# Autodesk Inventor assembly: Assieme_Disco
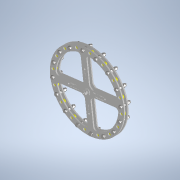
[picture p0: Inventor's stored thumbnail of the model, 180x180]
Saved by Autodesk Inventor 2020.2 (Build 242310000, 310)
## iProperties
Created: 2019-12-29
Part Number: Assieme_Disco
Document SubType Name: Assembly
Designer: socci
Mass: 580.168 g
Surface Area: 1810.87 cm^2
Volume: 239.955 cm^3
Density: 2.41782 g/cm^3
Author: socci
## Documents named in this file (8)
- C:\Users\socci\Desktop\mv-Project\04_PartDraw\Assieme_Disco.iam
- C:\Users\socci\Desktop\04_PartDraw\Componenti\24_Disco.ipt
- C:\Users\socci\Desktop\mv-Project\04_PartDraw\Componenti\26_Collana_di_Sfere.ipt
- C:\Users\socci\Documents\Inventor\Content Center Files\R2020\it-IT\DIN 1587\DIN 1587 - M6 x 1.ipt
- C:\Users\socci\Documents\Inventor\Content Center Files\R2020\it-IT\DIN 934\DIN 934 - M6 x 1.ipt
- C:\Users\socci\Desktop\mv-Project\04_PartDraw\Componenti\28_Rondella_M6.ipt
- C:\Users\socci\Documents\Inventor\Content Center Files\R2020\it-IT\DIN 933\DIN 933 - M6  x 30.ipt
- C:\Users\socci\Desktop\mv-Project\04_PartDraw\Componenti\9_Flangia.ipt
## Components (148 placed, 7 different names)
1. 24_Disco:1 — Inserimento:1, Inserimento:2, Inserimento:3, Inserimento:4
2. 24_Disco:2 — Inserimento:1, Inserimento:2, Inserimento:3, Inserimento:4, Coincidente:1, Coincidente:2, Inserimento:21, Inserimento:134, Inserimento:135, Coincidente:3, Inserimento:136, Inserimento:137, Inserimento:138, Inserimento:139, Inserimento:140, Inserimento:141, Inserimento:142, Inserimento:143, Inserimento:144, Inserimento:145, Inserimento:146, Inserimento:147, Inserimento:148, Coincidente:4, Inserimento:149, Inserimento:150
3. 26_Collana_di_Sfere:1 — Coincidente:1, Coincidente:2
4. DIN 933 - sostituito da DIN EN 24017 M6  x 30:1 — Inserimento:5
5. DIN 934 - sostituito da DIN EN 24032/28673/28674 M6:1 — Inserimento:7, Inserimento:8
6. 28_Rondella_M6:1 — Inserimento:5, Inserimento:6, Inserimento:134
7. 28_Rondella_M6:2 — Inserimento:6, Inserimento:7
8. 28_Rondella_M6:3 — Inserimento:8, Inserimento:9
9. 28_Rondella_M6:4 — Inserimento:11, Inserimento:12
10. 28_Rondella_M6:5 — Inserimento:9, Inserimento:10
11. 28_Rondella_M6:6 — Inserimento:10, Inserimento:11
12. DIN 1587 M6:1 — Inserimento:12
13. DIN 1587 M6:2
14. DIN 934 - sostituito da DIN EN 24032/28673/28674 M6:2
15. 28_Rondella_M6:7 — Inserimento:21
16. DIN 933 - sostituito da DIN EN 24017 M6  x 30:2
17. 28_Rondella_M6:8
18. 28_Rondella_M6:9
19. 28_Rondella_M6:10
20. 28_Rondella_M6:11
21. 28_Rondella_M6:12
22. DIN 1587 M6:3
23. DIN 934 - sostituito da DIN EN 24032/28673/28674 M6:3
24. 28_Rondella_M6:13 — Inserimento:147
25. DIN 933 - sostituito da DIN EN 24017 M6  x 30:3
26. 28_Rondella_M6:14
27. 28_Rondella_M6:15
28. 28_Rondella_M6:16
29. 28_Rondella_M6:17
30. 28_Rondella_M6:18
31. DIN 1587 M6:4
32. DIN 934 - sostituito da DIN EN 24032/28673/28674 M6:4
33. 28_Rondella_M6:19 — Inserimento:136
34. DIN 933 - sostituito da DIN EN 24017 M6  x 30:4
35. 28_Rondella_M6:20
36. 28_Rondella_M6:21
37. 28_Rondella_M6:22
38. 28_Rondella_M6:23
39. 28_Rondella_M6:24
40. DIN 1587 M6:5
41. DIN 934 - sostituito da DIN EN 24032/28673/28674 M6:5
42. 28_Rondella_M6:25 — Inserimento:146
43. DIN 933 - sostituito da DIN EN 24017 M6  x 30:5
44. 28_Rondella_M6:26
45. 28_Rondella_M6:27
46. 28_Rondella_M6:28
47. 28_Rondella_M6:29
48. 28_Rondella_M6:30
49. DIN 1587 M6:6
50. DIN 934 - sostituito da DIN EN 24032/28673/28674 M6:6
51. 28_Rondella_M6:31 — Inserimento:148
52. DIN 933 - sostituito da DIN EN 24017 M6  x 30:6
53. 28_Rondella_M6:32
54. 28_Rondella_M6:33
55. 28_Rondella_M6:34
56. 28_Rondella_M6:35
57. 28_Rondella_M6:36
58. DIN 1587 M6:7
59. DIN 934 - sostituito da DIN EN 24032/28673/28674 M6:7
60. 28_Rondella_M6:37 — Inserimento:144
61. DIN 933 - sostituito da DIN EN 24017 M6  x 30:7
62. 28_Rondella_M6:38
63. 28_Rondella_M6:39
64. 28_Rondella_M6:40
65. 28_Rondella_M6:41
66. 28_Rondella_M6:42
67. DIN 1587 M6:8
68. DIN 934 - sostituito da DIN EN 24032/28673/28674 M6:8
69. 28_Rondella_M6:43 — Inserimento:137
70. DIN 933 - sostituito da DIN EN 24017 M6  x 30:8
71. 28_Rondella_M6:44
72. 28_Rondella_M6:45
73. 28_Rondella_M6:46
74. 28_Rondella_M6:47
75. 28_Rondella_M6:48
76. DIN 1587 M6:9
77. DIN 934 - sostituito da DIN EN 24032/28673/28674 M6:9
78. 28_Rondella_M6:49 — Inserimento:138
79. DIN 933 - sostituito da DIN EN 24017 M6  x 30:9
80. 28_Rondella_M6:50
81. 28_Rondella_M6:51
82. 28_Rondella_M6:52
83. 28_Rondella_M6:53
84. 28_Rondella_M6:54
85. DIN 1587 M6:10
86. DIN 934 - sostituito da DIN EN 24032/28673/28674 M6:10
87. 28_Rondella_M6:55 — Inserimento:139
88. DIN 933 - sostituito da DIN EN 24017 M6  x 30:10
89. 28_Rondella_M6:56
90. 28_Rondella_M6:57
91. 28_Rondella_M6:58
92. 28_Rondella_M6:59
93. 28_Rondella_M6:60
94. DIN 1587 M6:11
95. DIN 934 - sostituito da DIN EN 24032/28673/28674 M6:11
96. 28_Rondella_M6:61 — Inserimento:145
97. DIN 933 - sostituito da DIN EN 24017 M6  x 30:11
98. 28_Rondella_M6:62
99. 28_Rondella_M6:63
100. 28_Rondella_M6:64
101. 28_Rondella_M6:65
102. 28_Rondella_M6:66
103. DIN 1587 M6:12
104. DIN 934 - sostituito da DIN EN 24032/28673/28674 M6:12
105. 28_Rondella_M6:67 — Inserimento:140
106. DIN 933 - sostituito da DIN EN 24017 M6  x 30:12
107. 28_Rondella_M6:68
108. 28_Rondella_M6:69
109. 28_Rondella_M6:70
110. 28_Rondella_M6:71
111. 28_Rondella_M6:72
112. DIN 1587 M6:13
113. DIN 934 - sostituito da DIN EN 24032/28673/28674 M6:13
114. 28_Rondella_M6:73 — Inserimento:143
115. DIN 933 - sostituito da DIN EN 24017 M6  x 30:13
116. 28_Rondella_M6:74
117. 28_Rondella_M6:75
118. 28_Rondella_M6:76
119. 28_Rondella_M6:77
120. 28_Rondella_M6:78
121. DIN 1587 M6:14
122. DIN 934 - sostituito da DIN EN 24032/28673/28674 M6:14
123. 28_Rondella_M6:79 — Inserimento:141
124. DIN 933 - sostituito da DIN EN 24017 M6  x 30:14
125. 28_Rondella_M6:80
126. 28_Rondella_M6:81
127. 28_Rondella_M6:82
128. 28_Rondella_M6:83
129. 28_Rondella_M6:84
130. DIN 1587 M6:15
131. DIN 934 - sostituito da DIN EN 24032/28673/28674 M6:15
132. 28_Rondella_M6:85 — Inserimento:142
133. DIN 933 - sostituito da DIN EN 24017 M6  x 30:15
134. 28_Rondella_M6:86
135. 28_Rondella_M6:87
136. 28_Rondella_M6:88
137. 28_Rondella_M6:89
138. 28_Rondella_M6:90
139. DIN 1587 M6:16
140. DIN 934 - sostituito da DIN EN 24032/28673/28674 M6:16
141. 28_Rondella_M6:91 — Inserimento:135
142. DIN 933 - sostituito da DIN EN 24017 M6  x 30:16
143. 28_Rondella_M6:92
144. 28_Rondella_M6:93
145. 28_Rondella_M6:94
146. 28_Rondella_M6:95
147. 28_Rondella_M6:96
148. 9_Flangia:1 — Coincidente:4, Inserimento:149, Inserimento:150
## Relationships (154: Insert 150, Mate 4)
- Inserimento:1 (7.829 mm): 24_Disco:1 ↔ 24_Disco:2
- Inserimento:2 (7.829 mm): 24_Disco:1 ↔ 24_Disco:2
- Inserimento:3 (7.829 mm): 24_Disco:1 ↔ 24_Disco:2
- Inserimento:4 (7.829 mm): 24_Disco:1 ↔ 24_Disco:2
- Coincidente:1 [Mate]: 24_Disco:2 ↔ 26_Collana_di_Sfere:1
- Coincidente:2 [Mate]: 24_Disco:2 ↔ 26_Collana_di_Sfere:1
- Inserimento:5: DIN 933 - sostituito da DIN EN 24017 M6  x 30:1 ↔ 28_Rondella_M6:1
- Inserimento:6 (4 mm): 28_Rondella_M6:1 ↔ 28_Rondella_M6:2
- Inserimento:7: DIN 934 - sostituito da DIN EN 24032/28673/28674 M6:1 ↔ 28_Rondella_M6:2
- Inserimento:8: DIN 934 - sostituito da DIN EN 24032/28673/28674 M6:1 ↔ 28_Rondella_M6:3
- Inserimento:9 (4 mm): 28_Rondella_M6:3 ↔ 28_Rondella_M6:5
- Inserimento:10: 28_Rondella_M6:5 ↔ 28_Rondella_M6:6
- Inserimento:11: 28_Rondella_M6:4 ↔ 28_Rondella_M6:6
- Inserimento:12: 28_Rondella_M6:4 ↔ DIN 1587 M6:1
- [Insert]: 28_Rondella_M6:7 ↔ DIN 933 - sostituito da DIN EN 24017 M6  x 30:2
- [Insert] (4 mm): 28_Rondella_M6:7 ↔ 28_Rondella_M6:8
- [Insert]: DIN 934 - sostituito da DIN EN 24032/28673/28674 M6:2 ↔ 28_Rondella_M6:8
- [Insert]: DIN 934 - sostituito da DIN EN 24032/28673/28674 M6:2 ↔ 28_Rondella_M6:9
- [Insert] (4 mm): 28_Rondella_M6:9 ↔ 28_Rondella_M6:11
- [Insert]: 28_Rondella_M6:11 ↔ 28_Rondella_M6:12
- [Insert]: 28_Rondella_M6:10 ↔ 28_Rondella_M6:12
- [Insert]: DIN 1587 M6:2 ↔ 28_Rondella_M6:10
- Inserimento:21: 24_Disco:2 ↔ 28_Rondella_M6:7
- [Insert]: 28_Rondella_M6:13 ↔ DIN 933 - sostituito da DIN EN 24017 M6  x 30:3
- [Insert] (4 mm): 28_Rondella_M6:13 ↔ 28_Rondella_M6:14
- [Insert]: DIN 934 - sostituito da DIN EN 24032/28673/28674 M6:3 ↔ 28_Rondella_M6:14
- [Insert]: DIN 934 - sostituito da DIN EN 24032/28673/28674 M6:3 ↔ 28_Rondella_M6:15
- [Insert] (4 mm): 28_Rondella_M6:15 ↔ 28_Rondella_M6:17
- [Insert]: 28_Rondella_M6:17 ↔ 28_Rondella_M6:18
- [Insert]: 28_Rondella_M6:16 ↔ 28_Rondella_M6:18
- [Insert]: DIN 1587 M6:3 ↔ 28_Rondella_M6:16
- [Insert]: 28_Rondella_M6:19 ↔ DIN 933 - sostituito da DIN EN 24017 M6  x 30:4
- [Insert] (4 mm): 28_Rondella_M6:19 ↔ 28_Rondella_M6:20
- [Insert]: DIN 934 - sostituito da DIN EN 24032/28673/28674 M6:4 ↔ 28_Rondella_M6:20
- [Insert]: DIN 934 - sostituito da DIN EN 24032/28673/28674 M6:4 ↔ 28_Rondella_M6:21
- [Insert] (4 mm): 28_Rondella_M6:21 ↔ 28_Rondella_M6:23
- [Insert]: 28_Rondella_M6:23 ↔ 28_Rondella_M6:24
- [Insert]: 28_Rondella_M6:22 ↔ 28_Rondella_M6:24
- [Insert]: DIN 1587 M6:4 ↔ 28_Rondella_M6:22
- [Insert]: 28_Rondella_M6:25 ↔ DIN 933 - sostituito da DIN EN 24017 M6  x 30:5
- [Insert] (4 mm): 28_Rondella_M6:25 ↔ 28_Rondella_M6:26
- [Insert]: DIN 934 - sostituito da DIN EN 24032/28673/28674 M6:5 ↔ 28_Rondella_M6:26
- [Insert]: DIN 934 - sostituito da DIN EN 24032/28673/28674 M6:5 ↔ 28_Rondella_M6:27
- [Insert] (4 mm): 28_Rondella_M6:27 ↔ 28_Rondella_M6:29
- [Insert]: 28_Rondella_M6:29 ↔ 28_Rondella_M6:30
- [Insert]: 28_Rondella_M6:28 ↔ 28_Rondella_M6:30
- [Insert]: DIN 1587 M6:5 ↔ 28_Rondella_M6:28
- [Insert]: 28_Rondella_M6:31 ↔ DIN 933 - sostituito da DIN EN 24017 M6  x 30:6
- [Insert] (4 mm): 28_Rondella_M6:31 ↔ 28_Rondella_M6:32
- [Insert]: DIN 934 - sostituito da DIN EN 24032/28673/28674 M6:6 ↔ 28_Rondella_M6:32
- [Insert]: DIN 934 - sostituito da DIN EN 24032/28673/28674 M6:6 ↔ 28_Rondella_M6:33
- [Insert] (4 mm): 28_Rondella_M6:33 ↔ 28_Rondella_M6:35
- [Insert]: 28_Rondella_M6:35 ↔ 28_Rondella_M6:36
- [Insert]: 28_Rondella_M6:34 ↔ 28_Rondella_M6:36
- [Insert]: DIN 1587 M6:6 ↔ 28_Rondella_M6:34
- [Insert]: 28_Rondella_M6:37 ↔ DIN 933 - sostituito da DIN EN 24017 M6  x 30:7
- [Insert] (4 mm): 28_Rondella_M6:37 ↔ 28_Rondella_M6:38
- [Insert]: DIN 934 - sostituito da DIN EN 24032/28673/28674 M6:7 ↔ 28_Rondella_M6:38
- [Insert]: DIN 934 - sostituito da DIN EN 24032/28673/28674 M6:7 ↔ 28_Rondella_M6:39
- [Insert] (4 mm): 28_Rondella_M6:39 ↔ 28_Rondella_M6:41
- [Insert]: 28_Rondella_M6:41 ↔ 28_Rondella_M6:42
- [Insert]: 28_Rondella_M6:40 ↔ 28_Rondella_M6:42
- [Insert]: DIN 1587 M6:7 ↔ 28_Rondella_M6:40
- [Insert]: 28_Rondella_M6:43 ↔ DIN 933 - sostituito da DIN EN 24017 M6  x 30:8
- [Insert] (4 mm): 28_Rondella_M6:43 ↔ 28_Rondella_M6:44
- [Insert]: DIN 934 - sostituito da DIN EN 24032/28673/28674 M6:8 ↔ 28_Rondella_M6:44
- [Insert]: DIN 934 - sostituito da DIN EN 24032/28673/28674 M6:8 ↔ 28_Rondella_M6:45
- [Insert] (4 mm): 28_Rondella_M6:45 ↔ 28_Rondella_M6:47
- [Insert]: 28_Rondella_M6:47 ↔ 28_Rondella_M6:48
- [Insert]: 28_Rondella_M6:46 ↔ 28_Rondella_M6:48
- [Insert]: DIN 1587 M6:8 ↔ 28_Rondella_M6:46
- [Insert]: 28_Rondella_M6:49 ↔ DIN 933 - sostituito da DIN EN 24017 M6  x 30:9
- [Insert] (4 mm): 28_Rondella_M6:49 ↔ 28_Rondella_M6:50
- [Insert]: DIN 934 - sostituito da DIN EN 24032/28673/28674 M6:9 ↔ 28_Rondella_M6:50
- [Insert]: DIN 934 - sostituito da DIN EN 24032/28673/28674 M6:9 ↔ 28_Rondella_M6:51
- [Insert] (4 mm): 28_Rondella_M6:51 ↔ 28_Rondella_M6:53
- [Insert]: 28_Rondella_M6:53 ↔ 28_Rondella_M6:54
- [Insert]: 28_Rondella_M6:52 ↔ 28_Rondella_M6:54
- [Insert]: DIN 1587 M6:9 ↔ 28_Rondella_M6:52
- [Insert]: 28_Rondella_M6:55 ↔ DIN 933 - sostituito da DIN EN 24017 M6  x 30:10
- [Insert] (4 mm): 28_Rondella_M6:55 ↔ 28_Rondella_M6:56
- [Insert]: DIN 934 - sostituito da DIN EN 24032/28673/28674 M6:10 ↔ 28_Rondella_M6:56
- [Insert]: DIN 934 - sostituito da DIN EN 24032/28673/28674 M6:10 ↔ 28_Rondella_M6:57
- [Insert] (4 mm): 28_Rondella_M6:57 ↔ 28_Rondella_M6:59
- [Insert]: 28_Rondella_M6:59 ↔ 28_Rondella_M6:60
- [Insert]: 28_Rondella_M6:58 ↔ 28_Rondella_M6:60
- [Insert]: DIN 1587 M6:10 ↔ 28_Rondella_M6:58
- [Insert]: 28_Rondella_M6:61 ↔ DIN 933 - sostituito da DIN EN 24017 M6  x 30:11
- [Insert] (4 mm): 28_Rondella_M6:61 ↔ 28_Rondella_M6:62
- [Insert]: DIN 934 - sostituito da DIN EN 24032/28673/28674 M6:11 ↔ 28_Rondella_M6:62
- [Insert]: DIN 934 - sostituito da DIN EN 24032/28673/28674 M6:11 ↔ 28_Rondella_M6:63
- [Insert] (4 mm): 28_Rondella_M6:63 ↔ 28_Rondella_M6:65
- [Insert]: 28_Rondella_M6:65 ↔ 28_Rondella_M6:66
- [Insert]: 28_Rondella_M6:64 ↔ 28_Rondella_M6:66
- [Insert]: DIN 1587 M6:11 ↔ 28_Rondella_M6:64
- [Insert]: 28_Rondella_M6:67 ↔ DIN 933 - sostituito da DIN EN 24017 M6  x 30:12
- [Insert] (4 mm): 28_Rondella_M6:67 ↔ 28_Rondella_M6:68
- [Insert]: DIN 934 - sostituito da DIN EN 24032/28673/28674 M6:12 ↔ 28_Rondella_M6:68
- [Insert]: DIN 934 - sostituito da DIN EN 24032/28673/28674 M6:12 ↔ 28_Rondella_M6:69
- [Insert] (4 mm): 28_Rondella_M6:69 ↔ 28_Rondella_M6:71
- [Insert]: 28_Rondella_M6:71 ↔ 28_Rondella_M6:72
- [Insert]: 28_Rondella_M6:70 ↔ 28_Rondella_M6:72
- [Insert]: DIN 1587 M6:12 ↔ 28_Rondella_M6:70
- [Insert]: 28_Rondella_M6:73 ↔ DIN 933 - sostituito da DIN EN 24017 M6  x 30:13
- [Insert] (4 mm): 28_Rondella_M6:73 ↔ 28_Rondella_M6:74
- [Insert]: DIN 934 - sostituito da DIN EN 24032/28673/28674 M6:13 ↔ 28_Rondella_M6:74
- [Insert]: DIN 934 - sostituito da DIN EN 24032/28673/28674 M6:13 ↔ 28_Rondella_M6:75
- [Insert] (4 mm): 28_Rondella_M6:75 ↔ 28_Rondella_M6:77
- [Insert]: 28_Rondella_M6:77 ↔ 28_Rondella_M6:78
- [Insert]: 28_Rondella_M6:76 ↔ 28_Rondella_M6:78
- [Insert]: DIN 1587 M6:13 ↔ 28_Rondella_M6:76
- [Insert]: 28_Rondella_M6:79 ↔ DIN 933 - sostituito da DIN EN 24017 M6  x 30:14
- [Insert] (4 mm): 28_Rondella_M6:79 ↔ 28_Rondella_M6:80
- [Insert]: DIN 934 - sostituito da DIN EN 24032/28673/28674 M6:14 ↔ 28_Rondella_M6:80
- [Insert]: DIN 934 - sostituito da DIN EN 24032/28673/28674 M6:14 ↔ 28_Rondella_M6:81
- [Insert] (4 mm): 28_Rondella_M6:81 ↔ 28_Rondella_M6:83
- [Insert]: 28_Rondella_M6:83 ↔ 28_Rondella_M6:84
- [Insert]: 28_Rondella_M6:82 ↔ 28_Rondella_M6:84
- [Insert]: DIN 1587 M6:14 ↔ 28_Rondella_M6:82
- [Insert]: 28_Rondella_M6:85 ↔ DIN 933 - sostituito da DIN EN 24017 M6  x 30:15
- [Insert] (4 mm): 28_Rondella_M6:85 ↔ 28_Rondella_M6:86
- [Insert]: DIN 934 - sostituito da DIN EN 24032/28673/28674 M6:15 ↔ 28_Rondella_M6:86
- [Insert]: DIN 934 - sostituito da DIN EN 24032/28673/28674 M6:15 ↔ 28_Rondella_M6:87
- [Insert] (4 mm): 28_Rondella_M6:87 ↔ 28_Rondella_M6:89
- [Insert]: 28_Rondella_M6:89 ↔ 28_Rondella_M6:90
- [Insert]: 28_Rondella_M6:88 ↔ 28_Rondella_M6:90
- [Insert]: DIN 1587 M6:15 ↔ 28_Rondella_M6:88
- [Insert]: 28_Rondella_M6:91 ↔ DIN 933 - sostituito da DIN EN 24017 M6  x 30:16
- [Insert] (4 mm): 28_Rondella_M6:91 ↔ 28_Rondella_M6:92
- [Insert]: DIN 934 - sostituito da DIN EN 24032/28673/28674 M6:16 ↔ 28_Rondella_M6:92
- [Insert]: DIN 934 - sostituito da DIN EN 24032/28673/28674 M6:16 ↔ 28_Rondella_M6:93
- [Insert] (4 mm): 28_Rondella_M6:93 ↔ 28_Rondella_M6:95
- [Insert]: 28_Rondella_M6:95 ↔ 28_Rondella_M6:96
- [Insert]: 28_Rondella_M6:94 ↔ 28_Rondella_M6:96
- [Insert]: DIN 1587 M6:16 ↔ 28_Rondella_M6:94
- Inserimento:134: 24_Disco:2 ↔ 28_Rondella_M6:1
- Inserimento:135: 24_Disco:2 ↔ 28_Rondella_M6:91
- Coincidente:3 [Mate]: 24_Disco:2
- Inserimento:136: 24_Disco:2 ↔ 28_Rondella_M6:19
- Inserimento:137: 24_Disco:2 ↔ 28_Rondella_M6:43
- Inserimento:138: 24_Disco:2 ↔ 28_Rondella_M6:49
- Inserimento:139: 24_Disco:2 ↔ 28_Rondella_M6:55
- Inserimento:140: 24_Disco:2 ↔ 28_Rondella_M6:67
- Inserimento:141: 24_Disco:2 ↔ 28_Rondella_M6:79
- Inserimento:142: 24_Disco:2 ↔ 28_Rondella_M6:85
- Inserimento:143: 24_Disco:2 ↔ 28_Rondella_M6:73
- Inserimento:144: 24_Disco:2 ↔ 28_Rondella_M6:37
- Inserimento:145: 24_Disco:2 ↔ 28_Rondella_M6:61
- Inserimento:146: 24_Disco:2 ↔ 28_Rondella_M6:25
- Inserimento:147: 24_Disco:2 ↔ 28_Rondella_M6:13
- Inserimento:148: 24_Disco:2 ↔ 28_Rondella_M6:31
- Coincidente:4 [Mate]: 24_Disco:2 ↔ 9_Flangia:1
- Inserimento:149: 24_Disco:2 ↔ 9_Flangia:1
- Inserimento:150: 24_Disco:2 ↔ 9_Flangia:1
## Named parameters: d14_d6 = 0 mm, d15_d7 = 4 mm, d16_d8 = 0 mm, d17_d9 = 0 mm, d18_d10 = 4 mm, d19_d11 = 0 mm, d20_d12 = 0 mm, d21_d13 = 0 mm, d23_d6 = 0 mm, d24_d7 = 4 mm, d25_d8 = 0 mm, d26_d9 = 0 mm, d27_d10 = 4 mm, d28_d11 = 0 mm, d29_d12 = 0 mm, d30_d13 = 0 mm, d31_d6 = 0 mm, d32_d7 = 4 mm, d33_d8 = 0 mm, d34_d9 = 0 mm, d35_d10 = 4 mm, d36_d11 = 0 mm, d37_d12 = 0 mm, d38_d13 = 0 mm, d39_d6 = 0 mm, d40_d7 = 4 mm, d41_d8 = 0 mm, d42_d9 = 0 mm, d43_d10 = 4 mm, d44_d11 = 0 mm, d45_d12 = 0 mm, d46_d13 = 0 mm, d47_d6 = 0 mm, d48_d7 = 4 mm, d49_d8 = 0 mm, d50_d9 = 0 mm, d51_d10 = 4 mm, d52_d11 = 0 mm, d53_d12 = 0 mm, d54_d13 = 0 mm, d55_d6 = 0 mm, d56_d7 = 4 mm, d57_d8 = 0 mm, d58_d9 = 0 mm, d59_d10 = 4 mm, d60_d11 = 0 mm, d61_d12 = 0 mm, d62_d13 = 0 mm, d63_d6 = 0 mm, d64_d7 = 4 mm, d65_d8 = 0 mm, d66_d9 = 0 mm, d67_d10 = 4 mm, d68_d11 = 0 mm, d69_d12 = 0 mm, d70_d13 = 0 mm, d71_d6 = 0 mm, d72_d7 = 4 mm, d73_d8 = 0 mm, d74_d9 = 0 mm, d75_d10 = 4 mm, d76_d11 = 0 mm, d77_d12 = 0 mm, d78_d13 = 0 mm, d79_d6 = 0 mm, d80_d7 = 4 mm, d81_d8 = 0 mm, d82_d9 = 0 mm, d83_d10 = 4 mm, d84_d11 = 0 mm, d85_d12 = 0 mm, d86_d13 = 0 mm, d87_d6 = 0 mm, d88_d7 = 4 mm, d89_d8 = 0 mm, d90_d9 = 0 mm, d91_d10 = 4 mm, d92_d11 = 0 mm, d93_d12 = 0 mm, d94_d13 = 0 mm, d95_d6 = 0 mm, d96_d7 = 4 mm, d97_d8 = 0 mm, d98_d9 = 0 mm, d99_d10 = 4 mm, d100_d11 = 0 mm, d101_d12 = 0 mm, d102_d13 = 0 mm, d103_d6 = 0 mm, d104_d7 = 4 mm, d105_d8 = 0 mm, d106_d9 = 0 mm, d107_d10 = 4 mm, d108_d11 = 0 mm, d109_d12 = 0 mm, d110_d13 = 0 mm, d111_d6 = 0 mm, d112_d7 = 4 mm, d113_d8 = 0 mm, d114_d9 = 0 mm, d115_d10 = 4 mm, d116_d11 = 0 mm, d117_d12 = 0 mm, d118_d13 = 0 mm, d119_d6 = 0 mm, d120_d7 = 4 mm, d121_d8 = 0 mm, d122_d9 = 0 mm, d123_d10 = 4 mm, d124_d11 = 0 mm, d125_d12 = 0 mm, d126_d13 = 0 mm, d127_d6 = 0 mm, d128_d7 = 4 mm, d129_d8 = 0 mm, d130_d9 = 0 mm, d131_d10 = 4 mm, d132_d11 = 0 mm, d133_d12 = 0 mm, d134_d13 = 0 mm
